# Autodesk Inventor assembly: M&M Hopper Assembly
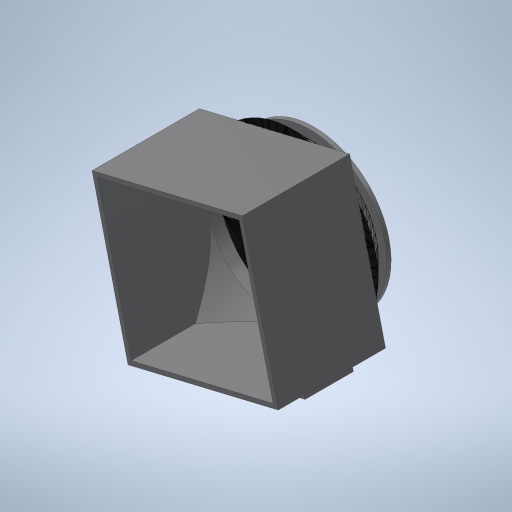
[picture p0: Inventor's stored thumbnail of the model, 512x512]
Saved by Autodesk Inventor 2023 (Build 270158000, 158)
## iProperties
Created: 2022-09-04
Part Number: M&M Hopper Assembly
Document SubType Name: Assembly
Designer: Garrett Raker
Title: Z:/ATMAE Robotics/Pill Dispenser Robot/Hoppers/M&M Hopper/M&M Hopper Assembly.step
## Documents named in this file (6)
- D:\College Stuff\ATMAE Robotics\Pill Dispenser Robot\Hoppers\Hopper Parts\Skittles Hopper Assembly.iam
- D:\College Stuff\ATMAE Robotics\Pill Dispenser Robot\Hoppers\Hopper Parts\Skate-Bearing v1.ipt
- D:\College Stuff\ATMAE Robotics\Pill Dispenser Robot\Hoppers\Hopper Parts\hopper bearing shaft v4.ipt
- D:\College Stuff\ATMAE Robotics\Pill Dispenser Robot\Hoppers\Hopper Parts\main Hopper body v6.ipt
- D:\College Stuff\ATMAE Robotics\Pill Dispenser Robot\Hoppers\Hopper Parts\Hopper baseplate lid thing v3.ipt
- D:\College Stuff\ATMAE Robotics\Pill Dispenser Robot\Hoppers\Dispensors\Skittles Dispensor.ipt
## Components (5 placed, 5 different names)
1. Skate-Bearing v1:1 — Mate:2, Mate:3
2. hopper bearing shaft v4:1 — Mate:1, Mate:2, Mate:4, Mate:6, Mate:7, Mate:9
3. main Hopper body v6:1 — Mate:3, Mate:4, Mate:5, Mate:7, Mate:8
4. Hopper baseplate lid thing v3:1 — Mate:6, Mate:8, Mate:9
5. Skittles Dispensor:1 — Mate:1, Mate:5
## Relationships (9: Mate 9)
- Mate:1: hopper bearing shaft v4:1 ↔ Skittles Dispensor:1
- Mate:2: Skate-Bearing v1:1 ↔ hopper bearing shaft v4:1
- Mate:3: Skate-Bearing v1:1 ↔ main Hopper body v6:1
- Mate:4: hopper bearing shaft v4:1 ↔ main Hopper body v6:1
- Mate:5: main Hopper body v6:1 ↔ Skittles Dispensor:1
- Mate:6: hopper bearing shaft v4:1 ↔ Hopper baseplate lid thing v3:1
- Mate:7: hopper bearing shaft v4:1 ↔ main Hopper body v6:1
- Mate:8: main Hopper body v6:1 ↔ Hopper baseplate lid thing v3:1
- Mate:9: hopper bearing shaft v4:1 ↔ Hopper baseplate lid thing v3:1
